# Autodesk Inventor assembly: BodyCupSketch
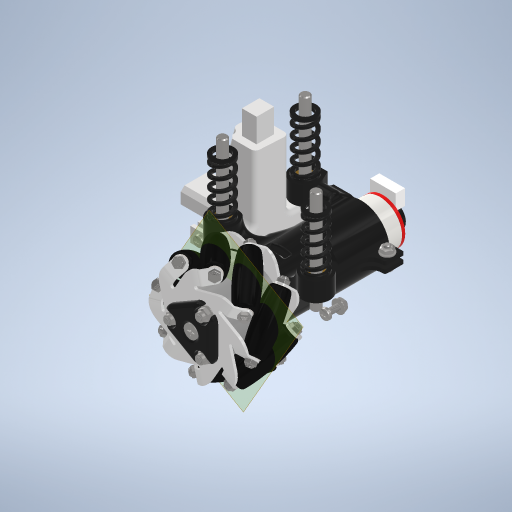
[picture p0: Inventor's stored thumbnail of the model, 512x512]
Saved by Autodesk Inventor 2023 (Build 270158000, 158)
## iProperties
Created: 2023-07-03
Part Number: BodyCupSketch
Document SubType Name: Assembly
Designer: khrip
Author: khrip
## Documents named in this file (8)
- C:\GoogleDrive\Cloud\Мой диск\Projects\Botik v0.1\BodyCupSketch.iam
- C:\GoogleDrive\Cloud\Мой диск\Projects\Botik v0.1\BodyCup.ipt
- C:\GoogleDrive\Cloud\Мой диск\Projects\Botik v0.1\suspensionUnit\suspensionUnit.iam
- C:\GoogleDrive\Cloud\Мой диск\Projects\Botik v0.1\spring v0.002.ipt
- C:\GoogleDrive\Cloud\Мой диск\Projects\Botik v0.1\axis.ipt
- C:\Users\khrip\Documents\Inventor\Content Center Files\R2023\ru-RU\BS EN ISO 7045 H\EN ISO 7045 - M3 x 10 - 4.8 - H(1).ipt
- C:\Users\khrip\Documents\Inventor\Content Center Files\R2023\ru-RU\GOST 11371-78  A\Шайба 3 ГОСТ 11371-78.ipt
- C:\Users\khrip\Documents\Inventor\Content Center Files\R2023\ru-RU\DIN 934\DIN 934 - M3 x 0,5.ipt
## Components (17 placed, 7 different names)
1. BodyCup:1 — Заподлицо:4, Совмещение:12, Совмещение:13, Совмещение:14, Совмещение:15, Совмещение:17, Совмещение:21, Совмещение:26, Совмещение:27, Совмещение:29
2. suspensionUnit:1 [sub-assembly] — Совмещение:1, Совмещение:2, Совмещение:3, Совмещение:4, Совмещение:5, Совмещение:6, Заподлицо:4
3. spring v0.002:1 — Совмещение:1, Совмещение:2, Совмещение:7, Заподлицо:1
4. spring v0.002:2 — Совмещение:4, Совмещение:6, Совмещение:8, Заподлицо:2
5. spring v0.002:3 — Совмещение:3, Совмещение:5, Совмещение:9, Заподлицо:3
6. axis:1 — Совмещение:7, Заподлицо:1
7. axis:2 — Совмещение:9, Заподлицо:3
8. axis:3 — Совмещение:8, Заподлицо:2
9. BS EN ISO 7045 H - метрическая M3 x 10 - 4.8 - H:1 — Совмещение:12, Совмещение:13, Совмещение:16, Совмещение:24
10. BS EN ISO 7045 H - метрическая M3 x 10 - 4.8 - H:2 — Совмещение:14, Совмещение:15, Совмещение:20, Совмещение:22
11. Шайба  ГОСТ 11371-78 3,2:1 — Совмещение:16, Совмещение:17, Совмещение:25
12. Шайба  ГОСТ 11371-78 3,2:2 — Совмещение:20, Совмещение:21, Совмещение:23
13. DIN 934 - заменено на DIN EN 24032/28673/28674 M3:1 — Совмещение:22, Совмещение:23
14. DIN 934 - заменено на DIN EN 24032/28673/28674 M3:2 — Совмещение:24, Совмещение:25
15. BS EN ISO 7045 H - метрическая M3 x 10 - 4.8 - H:3 — Совмещение:26, Совмещение:27, Совмещение:28, Совмещение:30
16. Шайба  ГОСТ 11371-78 3,2:3 — Совмещение:28, Совмещение:29, Совмещение:31
17. DIN 934 - заменено на DIN EN 24032/28673/28674 M3:3 — Совмещение:30, Совмещение:31
## Relationships (31: Mate 27, Flush 4)
- Совмещение:1 [Mate]: suspensionUnit:1 ↔ spring v0.002:1
- Совмещение:2 [Mate]: suspensionUnit:1 ↔ spring v0.002:1
- Совмещение:3 [Mate]: suspensionUnit:1 ↔ spring v0.002:3
- Совмещение:4 [Mate]: suspensionUnit:1 ↔ spring v0.002:2
- Совмещение:5 [Mate]: suspensionUnit:1 ↔ spring v0.002:3
- Совмещение:6 [Mate]: suspensionUnit:1 ↔ spring v0.002:2
- Совмещение:7 [Mate]: spring v0.002:1 ↔ axis:1
- Совмещение:8 [Mate]: spring v0.002:2 ↔ axis:3
- Совмещение:9 [Mate]: spring v0.002:3 ↔ axis:2
- Заподлицо:1 [Flush] (-8 mm): spring v0.002:1 ↔ axis:1
- Заподлицо:2 [Flush] (-8 mm): spring v0.002:2 ↔ axis:3
- Заподлицо:3 [Flush] (-8 mm): spring v0.002:3 ↔ axis:2
- Заподлицо:4 [Flush]: BodyCup:1 ↔ suspensionUnit:1
- Совмещение:12 [Mate]: BodyCup:1 ↔ BS EN ISO 7045 H - метрическая M3 x 10 - 4.8 - H:1
- Совмещение:13 [Mate]: BodyCup:1 ↔ BS EN ISO 7045 H - метрическая M3 x 10 - 4.8 - H:1
- Совмещение:14 [Mate]: BodyCup:1 ↔ BS EN ISO 7045 H - метрическая M3 x 10 - 4.8 - H:2
- Совмещение:15 [Mate]: BodyCup:1 ↔ BS EN ISO 7045 H - метрическая M3 x 10 - 4.8 - H:2
- Совмещение:16 [Mate]: BS EN ISO 7045 H - метрическая M3 x 10 - 4.8 - H:1 ↔ Шайба  ГОСТ 11371-78 3,2:1
- Совмещение:17 [Mate]: BodyCup:1 ↔ Шайба  ГОСТ 11371-78 3,2:1
- Совмещение:20 [Mate]: BS EN ISO 7045 H - метрическая M3 x 10 - 4.8 - H:2 ↔ Шайба  ГОСТ 11371-78 3,2:2
- Совмещение:21 [Mate]: BodyCup:1 ↔ Шайба  ГОСТ 11371-78 3,2:2
- Совмещение:22 [Mate]: BS EN ISO 7045 H - метрическая M3 x 10 - 4.8 - H:2 ↔ DIN 934 - заменено на DIN EN 24032/28673/28674 M3:1
- Совмещение:23 [Mate]: Шайба  ГОСТ 11371-78 3,2:2 ↔ DIN 934 - заменено на DIN EN 24032/28673/28674 M3:1
- Совмещение:24 [Mate]: BS EN ISO 7045 H - метрическая M3 x 10 - 4.8 - H:1 ↔ DIN 934 - заменено на DIN EN 24032/28673/28674 M3:2
- Совмещение:25 [Mate]: Шайба  ГОСТ 11371-78 3,2:1 ↔ DIN 934 - заменено на DIN EN 24032/28673/28674 M3:2
- Совмещение:26 [Mate]: BodyCup:1 ↔ BS EN ISO 7045 H - метрическая M3 x 10 - 4.8 - H:3
- Совмещение:27 [Mate]: BodyCup:1 ↔ BS EN ISO 7045 H - метрическая M3 x 10 - 4.8 - H:3
- Совмещение:28 [Mate]: BS EN ISO 7045 H - метрическая M3 x 10 - 4.8 - H:3 ↔ Шайба  ГОСТ 11371-78 3,2:3
- Совмещение:29 [Mate]: BodyCup:1 ↔ Шайба  ГОСТ 11371-78 3,2:3
- Совмещение:30 [Mate]: BS EN ISO 7045 H - метрическая M3 x 10 - 4.8 - H:3 ↔ DIN 934 - заменено на DIN EN 24032/28673/28674 M3:3
- Совмещение:31 [Mate]: Шайба  ГОСТ 11371-78 3,2:3 ↔ DIN 934 - заменено на DIN EN 24032/28673/28674 M3:3
